# Autodesk Inventor assembly: Onslaught V2
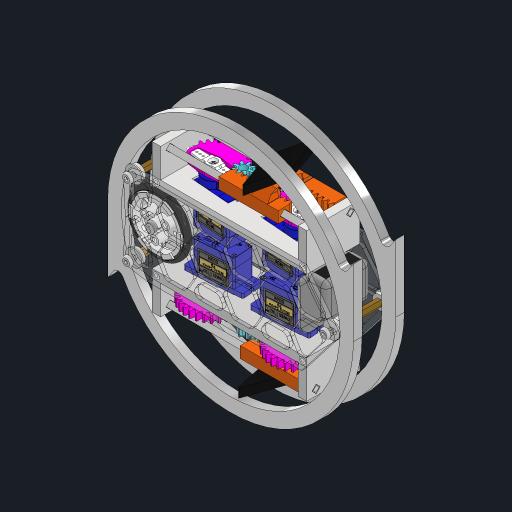
[picture p0: Inventor's stored thumbnail of the model, 512x512]
Saved by Autodesk Inventor 2023.2 (Build 272271030, 271C)
## iProperties
Created: 2024-02-26
Part Number: Onslaught V2
Document SubType Name: Assembly
Designer: robpl
Author: robpl
## Documents named in this file (9)
- C:\Users\robpl\OneDrive\Documents\Arduino\Onslaught\CAD\Onslaught V2.iam
- C:\Users\robpl\OneDrive\Documents\Arduino\Onslaught\CAD\Onslaught V2\Leg Module.iam
- C:\Users\robpl\OneDrive\Documents\Arduino\Onslaught\CAD\Ar620.ipt
- C:\Users\robpl\OneDrive\Documents\Arduino\Onslaught\CAD\BLHeli 12A ESC.ipt
- C:\Users\robpl\OneDrive\Documents\Arduino\Onslaught\CAD\Emax 1806 2280kv.ipt
- C:\Users\robpl\OneDrive\Documents\Arduino\Onslaught\CAD\Onslaught V2\Main Plate.ipt
- C:\Users\robpl\OneDrive\Documents\Arduino\Onslaught\CAD\tamiya-slim-tire-set-1.snapshot.2\36mm Slim Tamiya.iam
- C:\Users\robpl\OneDrive\Documents\Arduino\Onslaught\CAD\Onslaught V2\Bearing Assembly.iam
- C:\Users\robpl\OneDrive\Documents\Arduino\Onslaught\CAD\Onslaught V2\Ring.iam
## Components (12 placed, 8 different names)
1. Leg Module:1 [sub-assembly] — Flush:1, Flush:3, Flush:4, Mate:2, Flush:5, Mate:9, Mate:10, Mate:19, Mate:21
2. Leg Module:2 [sub-assembly] — Flush:1, Flush:6, Flush:7, Mate:7, Mate:8, Mate:11, Mate:20
3. Ar620:1 — Flush:3
4. BLHeli 12A ESC:1 — Flush:4, Mate:2, Flush:5
5. Emax 1806 2280kv:1 — Flush:6, Mate:5, Mate:6, Mate:12, Mate:13
6. Main Plate:1 — Mate:7, Mate:8, Mate:9, Mate:10, Mate:11, Mate:12, Mate:13, Mate:14, Mate:15, Mate:16, Mate:17, Mate:18
7. 36mm Slim Tamiya:1 [sub-assembly] — Mate:5, Mate:6
8. Bearing Assembly:1 [sub-assembly] — Flush:7, Mate:14, Tangent:2
9. Bearing Assembly:2 [sub-assembly] — Mate:17, Mate:18, Mate:22
10. Bearing Assembly:3 [sub-assembly] — Mate:15, Mate:16, Tangent:1
11. Main Plate:2 — Mate:19, Mate:20, Mate:21
12. Ring:1 [sub-assembly] — Mate:22, Tangent:1, Tangent:2
## Relationships (27: Mate 19, Flush 6, Tangent 2)
- Flush:1: Leg Module:1 ↔ Leg Module:2
- Flush:3: Leg Module:1 ↔ Ar620:1
- Flush:4: Leg Module:1 ↔ BLHeli 12A ESC:1
- Mate:2 (10 mm): Leg Module:1 ↔ BLHeli 12A ESC:1
- Flush:5 (20 mm): Leg Module:1 ↔ BLHeli 12A ESC:1
- Flush:6 (8 mm): Leg Module:2 ↔ Emax 1806 2280kv:1
- Mate:5: Emax 1806 2280kv:1 ↔ 36mm Slim Tamiya:1
- Mate:6: Emax 1806 2280kv:1 ↔ 36mm Slim Tamiya:1
- Flush:7: Leg Module:2 ↔ Bearing Assembly:1
- Mate:7: Leg Module:2 ↔ Main Plate:1
- Mate:8: Leg Module:2 ↔ Main Plate:1
- Mate:9: Leg Module:1 ↔ Main Plate:1
- Mate:10: Leg Module:1 ↔ Main Plate:1
- Mate:11: Leg Module:2 ↔ Main Plate:1
- Mate:12: Emax 1806 2280kv:1 ↔ Main Plate:1
- Mate:13: Emax 1806 2280kv:1 ↔ Main Plate:1
- Mate:14: Main Plate:1 ↔ Bearing Assembly:1
- Mate:15: Main Plate:1 ↔ Bearing Assembly:3
- Mate:16: Main Plate:1 ↔ Bearing Assembly:3
- Mate:17: Main Plate:1 ↔ Bearing Assembly:2
- Mate:18: Main Plate:1 ↔ Bearing Assembly:2
- Mate:19: Leg Module:1 ↔ Main Plate:2
- Mate:20: Leg Module:2 ↔ Main Plate:2
- Mate:21: Leg Module:1 ↔ Main Plate:2
- Mate:22: Bearing Assembly:2 ↔ Ring:1
- Tangent:1: Bearing Assembly:3 ↔ Ring:1
- Tangent:2: Bearing Assembly:1 ↔ Ring:1
